# Autodesk Inventor assembly: Pocketlab Voyager
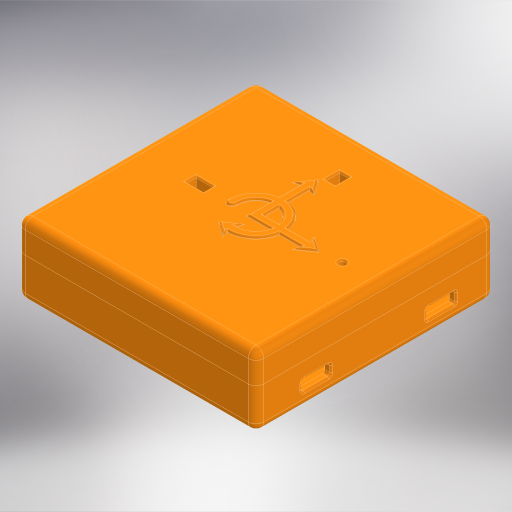
[picture p0: Inventor's stored thumbnail of the model, 512x512]
Saved by Autodesk Inventor 2024 (Build 280153000, 153)
## iProperties
Created: 2026-05-15
Part Number: Pocketlab Voyager
Document SubType Name: Assembly
Designer: Satyajit
Author: Satyajit
## Documents named in this file (4)
- C:\Users\Satyajit\Documents\Inventor\Swadhin\Pocket Lab voyager\Pocketlab Voyager.iam
- C:\Users\Satyajit\Documents\Inventor\Swadhin\Pocket Lab voyager\Bottom cover.ipt
- C:\Users\Satyajit\Documents\Inventor\Swadhin\Pocket Lab voyager\Top cover.ipt
- C:\Users\Satyajit\Documents\Inventor\Swadhin\Pocket Lab voyager\Logo.ipt
## Components (3 placed, 3 different names)
1. Bottom cover:1 — Rigid:1
2. Top cover:1 — Rigid:1, Rigid:2
3. Logo:1 — Rigid:2
## Relationships (2: WeldJoint 2)
- Rigid:1 [WeldJoint]: Bottom cover:1 ↔ Top cover:1
- Rigid:2 [WeldJoint]: Top cover:1 ↔ Logo:1
